# Autodesk Inventor assembly: Pierwsze podejscie
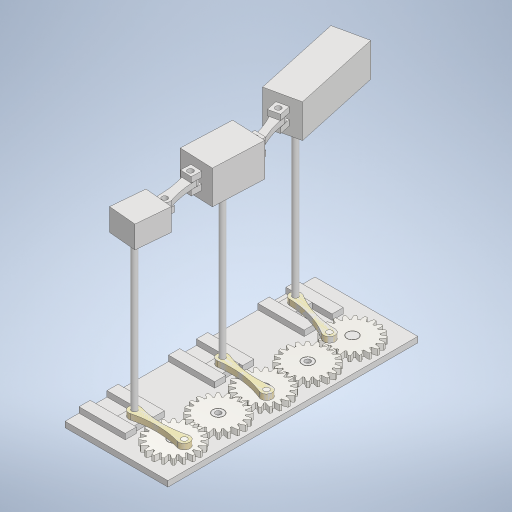
[picture p0: Inventor's stored thumbnail of the model, 512x512]
Saved by Autodesk Inventor 2024 (Build 280153000, 153)
## iProperties
Created: 2023-10-15
Part Number: Pierwsze podejscie
Document SubType Name: Assembly
Designer: Piter
Author: Piter
## Documents named in this file (13)
- C:\Users\Piter\OneDrive\Pulpit\Modele\Pierwsze podejscie.iam
- C:\Users\Piter\OneDrive\Pulpit\Modele\Podstawka.ipt
- C:\Users\Piter\OneDrive\Pulpit\Modele\suw.ipt
- C:\Users\Piter\OneDrive\Pulpit\Modele\support.ipt
- C:\Users\Piter\OneDrive\Pulpit\Modele\Pierwsze podejscie\Design Accelerator\Spur Gears3.iam
- C:\Users\Piter\OneDrive\Pulpit\Modele\Pierwsze podejscie\Design Accelerator\Spur Gears5.iam
- C:\Users\Piter\OneDrive\Pulpit\Modele\Pierwsze podejscie\Design Accelerator\Spur Gears6.iam
- C:\Users\Piter\OneDrive\Pulpit\Modele\Ramie.ipt
- C:\Users\Piter\OneDrive\Pulpit\Modele\head.ipt
- C:\Users\Piter\OneDrive\Pulpit\Modele\body.ipt
- C:\Users\Piter\OneDrive\Pulpit\Modele\body-connector.ipt
- C:\Users\Piter\OneDrive\Pulpit\Modele\tail.ipt
- C:\Users\Piter\OneDrive\Pulpit\Modele\body-tail.ipt
## Components (18 placed, 10 different names)
1. Podstawka:1 — Mate:7, Mate:8, Mate:13, Mate:16, Mate:31, Mate:33, Mate:35, Flush:1, Mate:36, Mate:37, Flush:2, Mate:38, Flush:3, Mate:39, Mate:44, Mate:45, Mate:51
2. suw:1 — Mate:7, Mate:8, Mate:40
3. suw:3 — Mate:13, Mate:16, Mate:50
4. support:1 — Mate:31, Mate:40, Mate:42, Mate:55, Mate:56
5. support:3 — Mate:33, Mate:46, Mate:47, Mate:57, Mate:58
6. Spur Gears:1 [sub-assembly] — Mate:35, Flush:1, Mate:36, Mate:41, Mate:43, Rotation:1
7. Spur Gears:2 [sub-assembly] — Mate:37, Flush:2, Mate:48, Mate:49, Rotation:1, Rotation:2
8. Spur Gears:3 [sub-assembly] — Mate:38, Flush:3, Mate:39, Mate:53, Mate:54, Rotation:2
9. Ramie:1 — Mate:41, Mate:42, Mate:43
10. suw:4 — Mate:44, Mate:45, Mate:46
11. Ramie:2 — Mate:47, Mate:48, Mate:49
12. support:4 — Mate:50, Mate:51, Mate:52, Mate:66, Mate:67
13. Ramie:3 — Mate:52, Mate:53, Mate:54
14. head:1 — Mate:55, Mate:56, Mate:61
15. body:1 — Mate:57, Mate:58, Mate:59, Mate:60, Mate:68, Mate:69
16. body-connector:1 — Mate:59, Mate:60, Mate:61
17. tail:1 — Mate:66, Mate:67, Mate:70
18. body-tail:1 — Mate:68, Mate:69, Mate:70
## Relationships (43: Mate 38, Flush 3, RelateRotation 2)
- Mate:7: Podstawka:1 ↔ suw:1
- Mate:8: Podstawka:1 ↔ suw:1
- Mate:13: Podstawka:1 ↔ suw:3
- Mate:16: Podstawka:1 ↔ suw:3
- Mate:31: Podstawka:1 ↔ support:1
- Mate:33: Podstawka:1 ↔ support:3
- Mate:35: Podstawka:1 ↔ Spur Gears:1
- Flush:1: Podstawka:1 ↔ Spur Gears:1
- Mate:36: Podstawka:1 ↔ Spur Gears:1
- Mate:37: Podstawka:1 ↔ Spur Gears:2
- Flush:2: Podstawka:1 ↔ Spur Gears:2
- Mate:38: Podstawka:1 ↔ Spur Gears:3
- Flush:3: Podstawka:1 ↔ Spur Gears:3
- Mate:39: Podstawka:1 ↔ Spur Gears:3
- Mate:40: suw:1 ↔ support:1
- Mate:41: Spur Gears:1 ↔ Ramie:1
- Mate:42: support:1 ↔ Ramie:1
- Mate:43: Spur Gears:1 ↔ Ramie:1
- Mate:44: Podstawka:1 ↔ suw:4
- Mate:45: Podstawka:1 ↔ suw:4
- Mate:46: support:3 ↔ suw:4
- Mate:47: support:3 ↔ Ramie:2
- Mate:48: Spur Gears:2 ↔ Ramie:2
- Mate:49: Spur Gears:2 ↔ Ramie:2
- Mate:50: suw:3 ↔ support:4
- Mate:51: Podstawka:1 ↔ support:4
- Mate:52: support:4 ↔ Ramie:3
- Mate:53: Spur Gears:3 ↔ Ramie:3
- Mate:54: Spur Gears:3 ↔ Ramie:3
- Mate:55: support:1 ↔ head:1
- Mate:56: support:1 ↔ head:1
- Mate:57: support:3 ↔ body:1
- Mate:58: support:3 ↔ body:1
- Mate:59: body:1 ↔ body-connector:1
- Mate:60: body:1 ↔ body-connector:1
- Mate:61: head:1 ↔ body-connector:1
- Mate:66: support:4 ↔ tail:1
- Mate:67: support:4 ↔ tail:1
- Mate:68: body:1 ↔ body-tail:1
- Mate:69: body:1 ↔ body-tail:1
- Mate:70: tail:1 ↔ body-tail:1
- Rotation:1 [RelateRotation] (1 ul): Spur Gears:1 ↔ Spur Gears:2
- Rotation:2 [RelateRotation] (1 ul): Spur Gears:2 ↔ Spur Gears:3
